# Autodesk Inventor assembly: Automoblox Assembly
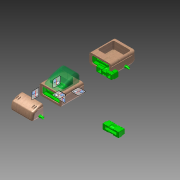
[picture p0: Inventor's stored thumbnail of the model, 180x180]
Saved by Autodesk Inventor 2015 (Build 190159000, 159)
## iProperties
Created: 2018-02-22
Part Number: Automoblox Assembly
Document SubType Name: Assembly
Designer: Administrator
Author: Administrator
## Documents named in this file (10)
- L:\IED 9th\Automoblox\7.4 Exact Parts\Automoblox Assembly.iam
- L:\IED 9th\Automoblox\7.4 Exact Parts\T9 Passenger Section.ipt
- L:\IED 9th\Automoblox\7.4 Exact Parts\T9 One Block Socket.ipt
- L:\IED 9th\Automoblox\7.4 Exact Parts\T9 Two Block Socket.ipt
- L:\IED 9th\Automoblox\7.4 Exact Parts\T9 Passenger Base.ipt
- L:\IED 9th\Automoblox\7.4 Exact Parts\T9 Connector.ipt
- L:\IED 9th\Automoblox\7.4 Exact Parts\T9 Windshield.ipt
- L:\IED 9th\Automoblox\7.4 Exact Parts\T9 Bed.ipt
- L:\IED 9th\Automoblox\7.4 Exact Parts\T9 Axle.ipt
- L:\IED 9th\Automoblox\7.4 Exact Parts\T9 Front.ipt
## Components (15 placed, 9 different names)
1. T9 Passenger Section:1 — Mate:7, Mate:8, Mate:9, Mate:10, Mate:11, Mate:12, Mate:13, Mate:14, Mate:15, Mate:16, Mate:17, Mate:18
2. T9 One Block Socket:1 — Mate:12, Mate:13, Mate:14
3. T9 One Block Socket:2 — Mate:19, Mate:20, Mate:21, Mate:25
4. T9 Two Block Socket:1 — Mate:7, Mate:8, Mate:15
5. T9 Two Block Socket:2 — Mate:22, Mate:23, Mate:24
6. T9 Passenger Base:1 — Mate:9, Mate:10, Mate:11
7. T9 Connector:1 — Mate:25
8. T9 Connector:2
9. T9 Windshield:1 — Mate:16, Mate:17, Mate:18
10. T9 Bed:1 — Mate:19, Mate:20, Mate:21, Insert:1, Insert:2
11. T9 Axle:1 — Insert:4
12. T9 Axle:2 — Insert:2
13. T9 Axle:3 — Insert:3
14. T9 Axle:4 — Insert:1
15. T9 Front:1 — Insert:3, Insert:4, Mate:22, Mate:23, Mate:24
## Relationships (23: Mate 19, Insert 4)
- Mate:7: T9 Passenger Section:1 ↔ T9 Two Block Socket:1
- Mate:8: T9 Passenger Section:1 ↔ T9 Two Block Socket:1
- Mate:9: T9 Passenger Section:1 ↔ T9 Passenger Base:1
- Mate:10: T9 Passenger Section:1 ↔ T9 Passenger Base:1
- Mate:11: T9 Passenger Section:1 ↔ T9 Passenger Base:1
- Mate:12: T9 Passenger Section:1 ↔ T9 One Block Socket:1
- Mate:13: T9 Passenger Section:1 ↔ T9 One Block Socket:1
- Mate:14: T9 Passenger Section:1 ↔ T9 One Block Socket:1
- Mate:15: T9 Passenger Section:1 ↔ T9 Two Block Socket:1
- Mate:16: T9 Passenger Section:1 ↔ T9 Windshield:1
- Mate:17: T9 Passenger Section:1 ↔ T9 Windshield:1
- Mate:18: T9 Passenger Section:1 ↔ T9 Windshield:1
- Mate:19: T9 One Block Socket:2 ↔ T9 Bed:1
- Mate:20: T9 One Block Socket:2 ↔ T9 Bed:1
- Mate:21: T9 One Block Socket:2 ↔ T9 Bed:1
- Insert:1: T9 Bed:1 ↔ T9 Axle:4
- Insert:2: T9 Bed:1 ↔ T9 Axle:2
- Insert:3: T9 Axle:3 ↔ T9 Front:1
- Insert:4: T9 Axle:1 ↔ T9 Front:1
- Mate:22: T9 Two Block Socket:2 ↔ T9 Front:1
- Mate:23: T9 Two Block Socket:2 ↔ T9 Front:1
- Mate:24: T9 Two Block Socket:2 ↔ T9 Front:1
- Mate:25: T9 One Block Socket:2 ↔ T9 Connector:1
